# Autodesk Inventor assembly: FE-00003
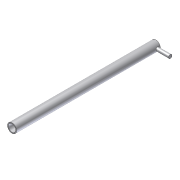
[picture p0: Inventor's stored thumbnail of the model, 180x180]
Saved by Autodesk Inventor 2012 (Build 160160000, 160)
## iProperties
Created: 2008-05-19
Part Number: FE-00003
Document SubType Name: Assembly
Designer: narosenberg
Author: narosenberg
## Documents named in this file (3)
- C:\Data Folder\FRC 2012 Field\Components\FE-00003.iam
- C:\Data Folder\FRC 2012 Field\Components\FE-00003-01.ipt
- C:\Data Folder\FRC 2012 Field\Components\FE-00003-02.ipt
## Components (2 placed, 2 different names)
1. FE-00003-01:1 — Mate:1, Tangent:1
2. FE-00003-02:1 — Mate:2, Tangent:1
## Relationships (4: Mate 3, Tangent 1)
- Mate:1: FE-00003-01:1
- Mate:2: FE-00003-02:1
- Mate:3
- Tangent:1 (-2.54 mm): FE-00003-01:1 ↔ FE-00003-02:1
